# Autodesk Inventor assembly: Assembly1
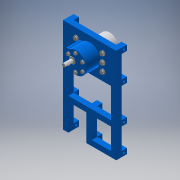
[picture p0: Inventor's stored thumbnail of the model, 180x180]
Saved by Autodesk Inventor 2016 (Build 200138000, 138)
## iProperties
Created: 2016-06-04
Part Number: Assembly1
Document SubType Name: Assembly
Designer: hesaon
Author: hesaon
## Documents named in this file (9)
- C:\Users\hesaon\Documents\Killer-Bot-2016\AutodeskWorkspace\robotparts revision 2\Assembly1.iam
- C:\Users\hesaon\Documents\Killer-Bot-2016\AutodeskWorkspace\robotparts revision 2\sideFrame.ipt
- C:\Users\hesaon\Documents\Killer-Bot-2016\AutodeskWorkspace\robotparts revision 2\motorHolder57mmVer2.ipt
- C:\Users\hesaon\Documents\Killer-Bot-2016\AutodeskWorkspace\robotparts revision 2\nut4mm.ipt
- C:\Users\hesaon\Documents\Killer-Bot-2016\AutodeskWorkspace\robotparts revision 2\screw18x4mm.ipt
- C:\Users\hesaon\Documents\Killer-Bot-2016\AutodeskWorkspace\robotparts revision 2\washer4mm.ipt
- C:\Users\hesaon\Documents\Killer-Bot-2016\AutodeskWorkspace\robotparts revision 2\37D mm metal gearmotor.ipt
- C:\Users\hesaon\Documents\Killer-Bot-2016\AutodeskWorkspace\robotparts revision 2\washer3mm.ipt
- C:\Users\hesaon\Documents\Killer-Bot-2016\AutodeskWorkspace\robotparts revision 2\screw12x3mm.ipt
## Components (39 placed, 8 different names)
1. sideFrame:1 — Insert:1, Insert:2, Insert:3, Insert:4, Insert:5, Insert:6, Insert:7, Insert:8
2. motorHolder57mmVer2:1 — Insert:1, Insert:2, Insert:9, Insert:10, Insert:11, Insert:12, Insert:13, Insert:14, Insert:27, Insert:28, Insert:29, Insert:30, Insert:31, Insert:32, Insert:33, Insert:34
3. nut4mm:1 — Insert:26
4. nut4mm:2 — Insert:21
5. nut4mm:3 — Insert:22
6. nut4mm:4 — Insert:23
7. nut4mm:5 — Insert:24
8. nut4mm:6 — Insert:25
9. screw18x4mm:1 — Insert:17
10. screw18x4mm:2 — Insert:19
11. screw18x4mm:3 — Insert:16
12. screw18x4mm:4 — Insert:15
13. screw18x4mm:5 — Insert:18
14. screw18x4mm:6 — Insert:20
15. washer4mm:1 — Insert:5, Insert:21
16. washer4mm:2 — Insert:8, Insert:24
17. washer4mm:3 — Insert:10, Insert:17
18. washer4mm:4 — Insert:9, Insert:15
19. washer4mm:5 — Insert:11, Insert:18
20. washer4mm:6 — Insert:12, Insert:19
21. washer4mm:7 — Insert:7, Insert:26
22. washer4mm:8 — Insert:13, Insert:16
23. washer4mm:9 — Insert:14, Insert:20
24. washer4mm:10 — Insert:4, Insert:23
25. washer4mm:11 — Insert:3, Insert:22
26. washer4mm:12 — Insert:6, Insert:25
27. 37D mm metal gearmotor:1 — Insert:27, Insert:28
28. washer3mm:1 — Insert:29, Insert:37
29. washer3mm:2 — Insert:30, Insert:36
30. washer3mm:3 — Insert:32, Insert:40
31. washer3mm:4 — Insert:31, Insert:35
32. washer3mm:5 — Insert:33, Insert:39
33. washer3mm:6 — Insert:34, Insert:38
34. screw12x3mm:1 — Insert:38
35. screw12x3mm:2 — Insert:35
36. screw12x3mm:3 — Insert:36
37. screw12x3mm:4 — Insert:37
38. screw12x3mm:5 — Insert:40
39. screw12x3mm:6 — Insert:39
## Relationships (40: Insert 40)
- Insert:1: sideFrame:1 ↔ motorHolder57mmVer2:1
- Insert:2: sideFrame:1 ↔ motorHolder57mmVer2:1
- Insert:3: sideFrame:1 ↔ washer4mm:11
- Insert:4: sideFrame:1 ↔ washer4mm:10
- Insert:5: sideFrame:1 ↔ washer4mm:1
- Insert:6: sideFrame:1 ↔ washer4mm:12
- Insert:7: sideFrame:1 ↔ washer4mm:7
- Insert:8: sideFrame:1 ↔ washer4mm:2
- Insert:9: motorHolder57mmVer2:1 ↔ washer4mm:4
- Insert:10: motorHolder57mmVer2:1 ↔ washer4mm:3
- Insert:11: motorHolder57mmVer2:1 ↔ washer4mm:5
- Insert:12: motorHolder57mmVer2:1 ↔ washer4mm:6
- Insert:13: motorHolder57mmVer2:1 ↔ washer4mm:8
- Insert:14: motorHolder57mmVer2:1 ↔ washer4mm:9
- Insert:15: screw18x4mm:4 ↔ washer4mm:4
- Insert:16: screw18x4mm:3 ↔ washer4mm:8
- Insert:17: screw18x4mm:1 ↔ washer4mm:3
- Insert:18: screw18x4mm:5 ↔ washer4mm:5
- Insert:19: screw18x4mm:2 ↔ washer4mm:6
- Insert:20: screw18x4mm:6 ↔ washer4mm:9
- Insert:21: nut4mm:2 ↔ washer4mm:1
- Insert:22: nut4mm:3 ↔ washer4mm:11
- Insert:23: nut4mm:4 ↔ washer4mm:10
- Insert:24: nut4mm:5 ↔ washer4mm:2
- Insert:25: nut4mm:6 ↔ washer4mm:12
- Insert:26: nut4mm:1 ↔ washer4mm:7
- Insert:27: motorHolder57mmVer2:1 ↔ 37D mm metal gearmotor:1
- Insert:28: motorHolder57mmVer2:1 ↔ 37D mm metal gearmotor:1
- Insert:29: motorHolder57mmVer2:1 ↔ washer3mm:1
- Insert:30: motorHolder57mmVer2:1 ↔ washer3mm:2
- Insert:31: motorHolder57mmVer2:1 ↔ washer3mm:4
- Insert:32: motorHolder57mmVer2:1 ↔ washer3mm:3
- Insert:33: motorHolder57mmVer2:1 ↔ washer3mm:5
- Insert:34: motorHolder57mmVer2:1 ↔ washer3mm:6
- Insert:35: washer3mm:4 ↔ screw12x3mm:2
- Insert:36: washer3mm:2 ↔ screw12x3mm:3
- Insert:37: washer3mm:1 ↔ screw12x3mm:4
- Insert:38: washer3mm:6 ↔ screw12x3mm:1
- Insert:39: washer3mm:5 ↔ screw12x3mm:6
- Insert:40: washer3mm:3 ↔ screw12x3mm:5
